# Autodesk Inventor assembly: RP-lidar-A1
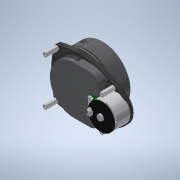
[picture p0: Inventor's stored thumbnail of the model, 180x180]
Saved by Autodesk Inventor 2021 (Build 250183000, 183)
## iProperties
Created: 2018-07-31
Part Number: RP-lidar-A1
Document SubType Name: Assembly
Designer: aespen-cad
Author: aespen-cad
## Documents named in this file (18)
- C:\Users\User\Desktop\Bachelorarbeit\CAD\RP-lidar-A1\RP-lidar-A1.iam
- C:\Users\User\Desktop\Bachelorarbeit\CAD\RP-lidar-A1\base.ipt
- C:\Users\User\Desktop\Bachelorarbeit\CAD\RP-lidar-A1\head-base.ipt
- C:\Users\User\Desktop\Bachelorarbeit\CAD\RP-lidar-A1\detector-mount.ipt
- C:\Users\User\Desktop\Bachelorarbeit\CAD\RP-lidar-A1\detector.ipt
- C:\Users\User\Desktop\Bachelorarbeit\CAD\RP-lidar-A1\laser.ipt
- C:\Users\User\Desktop\Bachelorarbeit\CAD\RP-lidar-A1\laser-mount.ipt
- C:\Users\User\Desktop\Bachelorarbeit\CAD\RP-lidar-A1\head.ipt
- C:\Users\User\Desktop\Bachelorarbeit\CAD\RP-lidar-A1\Woodscrews_GB_TYPE136 M2X6-N.ipt
- C:\Users\User\Desktop\Bachelorarbeit\CAD\RP-lidar-A1\motherboard.ipt
- C:\Users\User\Desktop\Bachelorarbeit\CAD\RP-lidar-A1\connector-1_25-3pin.ipt
- C:\Users\User\Desktop\Bachelorarbeit\CAD\RP-lidar-A1\motor.ipt
- C:\Users\User\Desktop\Bachelorarbeit\CAD\RP-lidar-A1\motor-board.ipt
- C:\Users\User\Desktop\Bachelorarbeit\CAD\RP-lidar-A1\connector-1_25-4pin.ipt
- C:\Users\User\Desktop\Bachelorarbeit\CAD\RP-lidar-A1\bottom-lid.ipt
- C:\Users\User\Desktop\Bachelorarbeit\CAD\RP-lidar-A1\stand_15x2.ipt
- C:\Users\User\Desktop\Bachelorarbeit\CAD\RP-lidar-A1\rubber.ipt
- C:\Users\User\Desktop\Bachelorarbeit\CAD\RP-lidar-A1\wheel.ipt
## Components (24 placed, 17 different names)
1. base:1 — Insert:8, Insert:9, Insert:11, Mate:7, Insert:12, Insert:13, Mate:8, Mate:9, Insert:16, Insert:17, Insert:18, Insert:19
2. head-base:1 — Mate:2, Mate:3, Insert:3, Insert:4, Mate:8, Mate:9, Mate:10, Mate:11, Angle:1
3. detector-mount:1 — Insert:1, Mate:2, Mate:3
4. detector:1 — Insert:1
5. laser:1 — Insert:2
6. laser-mount:1 — Insert:2, Mate:10, Mate:11, Angle:1
7. head:1 — Insert:3, Insert:4, Insert:5, Insert:6, Insert:7, Mate:15
8. Woodscrews_GB_TYPE136 M2X6-N:1 — Insert:5
9. Woodscrews_GB_TYPE136 M2X6-N:2 — Insert:7
10. Woodscrews_GB_TYPE136 M2X6-N:3 — Insert:6
11. motherboard:1 — Insert:8, Insert:9, Mate:13, Flush:3, Flush:4, Insert:14, Insert:15
12. connector-1_25-3pin:1 — Mate:12, Flush:1, Flush:2
13. motor:1 — Insert:10, Insert:11, Mate:7, Flush:1, Flush:2, Insert:28
14. motor-board:1 — Insert:10, Mate:12
15. Woodscrews_GB_TYPE136 M2X6-N:4 — Insert:13
16. Woodscrews_GB_TYPE136 M2X6-N:5 — Insert:12
17. connector-1_25-4pin:1 — Mate:13, Flush:3, Flush:4
18. bottom-lid:1 — Insert:14, Insert:15
19. stand_15x2:1 — Insert:19
20. stand_15x2:2 — Insert:18
21. stand_15x2:3 — Insert:17
22. stand_15x2:4 — Insert:16
23. rubber:1 — Mate:14, Mate:15
24. wheel:1 — Insert:28, Mate:14
## Relationships (36: Insert 20, Mate 11, Flush 4, Angle 1)
- Insert:1: detector-mount:1 ↔ detector:1
- Mate:2: head-base:1 ↔ detector-mount:1
- Mate:3: head-base:1 ↔ detector-mount:1
- Insert:2 (-5 mm): laser:1 ↔ laser-mount:1
- Insert:3: head-base:1 ↔ head:1
- Insert:4: head-base:1 ↔ head:1
- Insert:5: head:1 ↔ Woodscrews_GB_TYPE136 M2X6-N:1
- Insert:6: head:1 ↔ Woodscrews_GB_TYPE136 M2X6-N:3
- Insert:7: head:1 ↔ Woodscrews_GB_TYPE136 M2X6-N:2
- Insert:8: base:1 ↔ motherboard:1
- Insert:9: base:1 ↔ motherboard:1
- Insert:10: motor:1 ↔ motor-board:1
- Insert:11: base:1 ↔ motor:1
- Mate:7: base:1 ↔ motor:1
- Insert:12: base:1 ↔ Woodscrews_GB_TYPE136 M2X6-N:5
- Insert:13: base:1 ↔ Woodscrews_GB_TYPE136 M2X6-N:4
- Mate:8: base:1 ↔ head-base:1
- Mate:9: base:1 ↔ head-base:1
- Mate:10: head-base:1 ↔ laser-mount:1
- Mate:11: head-base:1 ↔ laser-mount:1
- Angle:1 (113.5 deg): head-base:1 ↔ laser-mount:1
- Mate:12: connector-1_25-3pin:1 ↔ motor-board:1
- Flush:1 (-14 mm): connector-1_25-3pin:1 ↔ motor:1
- Flush:2 (-11 mm): connector-1_25-3pin:1 ↔ motor:1
- Mate:13: motherboard:1 ↔ connector-1_25-4pin:1
- Flush:3 (23.5 mm): motherboard:1 ↔ connector-1_25-4pin:1
- Flush:4 (-4 mm): motherboard:1 ↔ connector-1_25-4pin:1
- Insert:14: motherboard:1 ↔ bottom-lid:1
- Insert:15: motherboard:1 ↔ bottom-lid:1
- Insert:16: base:1 ↔ stand_15x2:4
- Insert:17: base:1 ↔ stand_15x2:3
- Insert:18: base:1 ↔ stand_15x2:2
- Insert:19: base:1 ↔ stand_15x2:1
- Insert:28: motor:1 ↔ wheel:1
- Mate:14: rubber:1 ↔ wheel:1
- Mate:15: head:1 ↔ rubber:1
